# Autodesk Inventor assembly: Factions_Normal
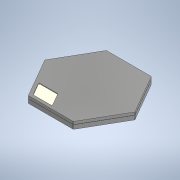
[picture p0: Inventor's stored thumbnail of the model, 180x180]
Saved by Autodesk Inventor 2021 (Build 250183000, 183)
## iProperties
Created: 2023-03-16
Part Number: Factions_Normal
Document SubType Name: Assembly
Designer: Bradley
Author: Bradley
## Documents named in this file (7)
- C:\Users\Bradley\Git\TI4\Factions\Factions_Normal.iam
- C:\Users\Bradley\Git\TI4\Components\Hex_Single.ipt
- C:\Users\Bradley\Git\TI4\Components\FactionCards_All.ipt
- C:\Users\Bradley\Git\TI4\Factions\Factions_Lid.ipt
- C:\Users\Bradley\Git\TI4\Factions\Factions_Base.ipt
- C:\Users\Bradley\Git\TI4\Components\CommandToken_Single.ipt
- C:\Users\Bradley\Git\TI4\Components\ControlMarker_Single.ipt
## Components (37 placed, 6 different names)
1. Factions_Base:1 — Mate:1, Flush:1, Flush:2, Mate:2, Mate:3, Mate:4, Mate:5, Mate:8, Mate:11, Mate:12, Mate:13, Mate:30, Mate:31, Mate:32, Mate:33, Mate:35, Mate:36, Mate:37, Mate:39, Mate:41, Mate:42, Mate:43, Mate:44, Mate:45, Mate:47, Mate:48, Mate:49, Mate:50, Mate:52, Mate:53, Mate:56, Mate:59, Mate:61
2. Factions_Lid:1 — Mate:1, Flush:1, Flush:2
3. CommandToken_Single:1 — Mate:6, Flush:6, Flush:8, Mate:8, Mate:12, Mate:13, Mate:60
4. CommandToken_Single:10 — Mate:36, Mate:37, Mate:38, Mate:40
5. CommandToken_Single:11
6. CommandToken_Single:12
7. CommandToken_Single:13 — Mate:39, Mate:40, Mate:41
8. CommandToken_Single:14
9. CommandToken_Single:15
10. CommandToken_Single:16 — Mate:58, Mate:61, Flush:47
11. CommandToken_Single:2 — Mate:6, Mate:7, Flush:5, Flush:6, Flush:7, Flush:8
12. CommandToken_Single:3 — Mate:7, Flush:5, Flush:7
13. CommandToken_Single:4 — Mate:30, Mate:31, Mate:32, Mate:34
14. CommandToken_Single:5
15. CommandToken_Single:6
16. CommandToken_Single:7 — Mate:33, Mate:34, Mate:35, Mate:38
17. CommandToken_Single:8
18. CommandToken_Single:9
19. ControlMarker_Single:1 — Mate:9, Flush:9, Flush:11, Mate:11, Mate:42, Mate:43, Mate:46
20. ControlMarker_Single:10 — Mate:47, Mate:48, Mate:49, Mate:51
21. ControlMarker_Single:11
22. ControlMarker_Single:12
23. ControlMarker_Single:13 — Mate:50, Mate:51, Mate:52, Mate:54
24. ControlMarker_Single:14
25. ControlMarker_Single:15
26. ControlMarker_Single:16 — Mate:56, Mate:57, Flush:45, Flush:46, Mate:59, Mate:60
27. ControlMarker_Single:17 — Mate:57, Mate:58, Flush:45, Flush:46, Flush:47
28. ControlMarker_Single:2 — Mate:9, Mate:10, Flush:9, Flush:10, Flush:11, Flush:12
29. ControlMarker_Single:3 — Mate:10, Flush:10, Flush:12
30. ControlMarker_Single:4 — Mate:53, Mate:54, Mate:55
31. ControlMarker_Single:5
32. ControlMarker_Single:6
33. ControlMarker_Single:7 — Mate:44, Mate:45, Mate:46, Mate:55
34. ControlMarker_Single:8
35. ControlMarker_Single:9
36. FactionCards_All:1 — Mate:3, Mate:4, Mate:5
37. Hex_Single:1 — Mate:2, Flush:3, Flush:4
## Relationships (108: Mate 61, Flush 47)
- Mate:1: Factions_Base:1 ↔ Factions_Lid:1
- Flush:1: Factions_Base:1 ↔ Factions_Lid:1
- Flush:2: Factions_Base:1 ↔ Factions_Lid:1
- Mate:2: Factions_Base:1 ↔ Hex_Single:1
- Flush:3: Hex_Single:1
- Flush:4: Hex_Single:1
- Mate:3: Factions_Base:1 ↔ FactionCards_All:1
- Mate:4 (0.5 mm): Factions_Base:1 ↔ FactionCards_All:1
- Mate:5 (0.5 mm): Factions_Base:1 ↔ FactionCards_All:1
- Mate:6: CommandToken_Single:1 ↔ CommandToken_Single:2
- Mate:7: CommandToken_Single:2 ↔ CommandToken_Single:3
- Flush:5: CommandToken_Single:2 ↔ CommandToken_Single:3
- Flush:6: CommandToken_Single:1 ↔ CommandToken_Single:2
- Flush:7: CommandToken_Single:2 ↔ CommandToken_Single:3
- Flush:8: CommandToken_Single:1 ↔ CommandToken_Single:2
- Mate:8: Factions_Base:1 ↔ CommandToken_Single:1
- Mate:9: ControlMarker_Single:1 ↔ ControlMarker_Single:2
- Mate:10: ControlMarker_Single:2 ↔ ControlMarker_Single:3
- Flush:9: ControlMarker_Single:1 ↔ ControlMarker_Single:2
- Flush:10: ControlMarker_Single:2 ↔ ControlMarker_Single:3
- Flush:11: ControlMarker_Single:1 ↔ ControlMarker_Single:2
- Flush:12: ControlMarker_Single:2 ↔ ControlMarker_Single:3
- Mate:11: Factions_Base:1 ↔ ControlMarker_Single:1
- Mate:12 (0.5 mm): Factions_Base:1 ↔ CommandToken_Single:1
- Mate:13 (0.5 mm): Factions_Base:1 ↔ CommandToken_Single:1
- [Mate]: CommandToken_Single:4 ↔ CommandToken_Single:5
- [Mate]: CommandToken_Single:5 ↔ CommandToken_Single:6
- [Flush]: CommandToken_Single:5 ↔ CommandToken_Single:6
- [Flush]: CommandToken_Single:4 ↔ CommandToken_Single:5
- [Flush]: CommandToken_Single:5 ↔ CommandToken_Single:6
- [Flush]: CommandToken_Single:4 ↔ CommandToken_Single:5
- [Mate]: CommandToken_Single:7 ↔ CommandToken_Single:8
- [Mate]: CommandToken_Single:8 ↔ CommandToken_Single:9
- [Flush]: CommandToken_Single:8 ↔ CommandToken_Single:9
- [Flush]: CommandToken_Single:7 ↔ CommandToken_Single:8
- [Flush]: CommandToken_Single:8 ↔ CommandToken_Single:9
- [Flush]: CommandToken_Single:7 ↔ CommandToken_Single:8
- [Mate]: CommandToken_Single:10 ↔ CommandToken_Single:11
- [Mate]: CommandToken_Single:11 ↔ CommandToken_Single:12
- [Flush]: CommandToken_Single:11 ↔ CommandToken_Single:12
- [Flush]: CommandToken_Single:10 ↔ CommandToken_Single:11
- [Flush]: CommandToken_Single:11 ↔ CommandToken_Single:12
- [Flush]: CommandToken_Single:10 ↔ CommandToken_Single:11
- [Mate]: CommandToken_Single:13 ↔ CommandToken_Single:14
- [Mate]: CommandToken_Single:14 ↔ CommandToken_Single:15
- [Flush]: CommandToken_Single:14 ↔ CommandToken_Single:15
- [Flush]: CommandToken_Single:13 ↔ CommandToken_Single:14
- [Flush]: CommandToken_Single:14 ↔ CommandToken_Single:15
- [Flush]: CommandToken_Single:13 ↔ CommandToken_Single:14
- [Mate]: ControlMarker_Single:4 ↔ ControlMarker_Single:5
- [Mate]: ControlMarker_Single:5 ↔ ControlMarker_Single:6
- [Flush]: ControlMarker_Single:4 ↔ ControlMarker_Single:5
- [Flush]: ControlMarker_Single:5 ↔ ControlMarker_Single:6
- [Flush]: ControlMarker_Single:4 ↔ ControlMarker_Single:5
- [Flush]: ControlMarker_Single:5 ↔ ControlMarker_Single:6
- [Mate]: ControlMarker_Single:7 ↔ ControlMarker_Single:8
- [Mate]: ControlMarker_Single:8 ↔ ControlMarker_Single:9
- [Flush]: ControlMarker_Single:7 ↔ ControlMarker_Single:8
- [Flush]: ControlMarker_Single:8 ↔ ControlMarker_Single:9
- [Flush]: ControlMarker_Single:7 ↔ ControlMarker_Single:8
- [Flush]: ControlMarker_Single:8 ↔ ControlMarker_Single:9
- [Mate]: ControlMarker_Single:10 ↔ ControlMarker_Single:11
- [Mate]: ControlMarker_Single:11 ↔ ControlMarker_Single:12
- [Flush]: ControlMarker_Single:10 ↔ ControlMarker_Single:11
- [Flush]: ControlMarker_Single:11 ↔ ControlMarker_Single:12
- [Flush]: ControlMarker_Single:10 ↔ ControlMarker_Single:11
- [Flush]: ControlMarker_Single:11 ↔ ControlMarker_Single:12
- [Mate]: ControlMarker_Single:13 ↔ ControlMarker_Single:14
- [Mate]: ControlMarker_Single:14 ↔ ControlMarker_Single:15
- [Flush]: ControlMarker_Single:13 ↔ ControlMarker_Single:14
- [Flush]: ControlMarker_Single:14 ↔ ControlMarker_Single:15
- [Flush]: ControlMarker_Single:13 ↔ ControlMarker_Single:14
- [Flush]: ControlMarker_Single:14 ↔ ControlMarker_Single:15
- Mate:30: Factions_Base:1 ↔ CommandToken_Single:4
- Mate:31 (0.5 mm): Factions_Base:1 ↔ CommandToken_Single:4
- Mate:32 (0.5 mm): Factions_Base:1 ↔ CommandToken_Single:4
- Mate:33: Factions_Base:1 ↔ CommandToken_Single:7
- Mate:34 (0.5 mm): CommandToken_Single:4 ↔ CommandToken_Single:7
- Mate:35 (0.5 mm): Factions_Base:1 ↔ CommandToken_Single:7
- Mate:36: Factions_Base:1 ↔ CommandToken_Single:10
- Mate:37 (0.5 mm): Factions_Base:1 ↔ CommandToken_Single:10
- Mate:38 (0.5 mm): CommandToken_Single:10 ↔ CommandToken_Single:7
- Mate:39: Factions_Base:1 ↔ CommandToken_Single:13
- Mate:40 (0.5 mm): CommandToken_Single:10 ↔ CommandToken_Single:13
- Mate:41 (0.5 mm): Factions_Base:1 ↔ CommandToken_Single:13
- Mate:42 (0.5 mm): Factions_Base:1 ↔ ControlMarker_Single:1
- Mate:43 (0.5 mm): Factions_Base:1 ↔ ControlMarker_Single:1
- Mate:44: Factions_Base:1 ↔ ControlMarker_Single:7
- Mate:45 (0.5 mm): Factions_Base:1 ↔ ControlMarker_Single:7
- Mate:46 (0.5 mm): ControlMarker_Single:1 ↔ ControlMarker_Single:7
- Mate:47: Factions_Base:1 ↔ ControlMarker_Single:10
- Mate:48 (0.5 mm): Factions_Base:1 ↔ ControlMarker_Single:10
- Mate:49 (0.5 mm): Factions_Base:1 ↔ ControlMarker_Single:10
- Mate:50: Factions_Base:1 ↔ ControlMarker_Single:13
- Mate:51 (0.5 mm): ControlMarker_Single:10 ↔ ControlMarker_Single:13
- Mate:52 (0.5 mm): Factions_Base:1 ↔ ControlMarker_Single:13
- Mate:53: Factions_Base:1 ↔ ControlMarker_Single:4
- Mate:54 (0.5 mm): ControlMarker_Single:13 ↔ ControlMarker_Single:4
- Mate:55: ControlMarker_Single:4 ↔ ControlMarker_Single:7
- Mate:56: Factions_Base:1 ↔ ControlMarker_Single:16
- Mate:57: ControlMarker_Single:16 ↔ ControlMarker_Single:17
- Mate:58: CommandToken_Single:16 ↔ ControlMarker_Single:17
- Flush:45: ControlMarker_Single:16 ↔ ControlMarker_Single:17
- Flush:46: ControlMarker_Single:16 ↔ ControlMarker_Single:17
- Mate:59 (0.5 mm): Factions_Base:1 ↔ ControlMarker_Single:16
- Mate:60 (0.5 mm): CommandToken_Single:1 ↔ ControlMarker_Single:16
- Mate:61 (0.5 mm): Factions_Base:1 ↔ CommandToken_Single:16
- Flush:47: CommandToken_Single:16 ↔ ControlMarker_Single:17
## Named parameters: d25_d14 = 0 mm, d26_d9 = 0 mm, d27_d10 = 0 mm, d28_d11 = 0 mm, d29_d12 = 0 mm, d30_d13 = 0 mm, d31_d14 = 0 mm, d32_d9 = 0 mm, d33_d10 = 0 mm, d34_d11 = 0 mm, d35_d12 = 0 mm, d36_d13 = 0 mm, d37_d14 = 0 mm, d38_d9 = 0 mm, d39_d10 = 0 mm, d40_d11 = 0 mm, d41_d12 = 0 mm, d42_d13 = 0 mm, d43_d14 = 0 mm, d44_d9 = 0 mm, d45_d10 = 0 mm, d46_d11 = 0 mm, d47_d12 = 0 mm, d48_d13 = 0 mm, d49_d16 = 0 mm, d50_d17 = 0 mm, d51_d18 = 0 mm, d52_d19 = 0 mm, d53_d20 = 0 mm, d54_d21 = 0 mm, d55_d16 = 0 mm, d56_d17 = 0 mm, d57_d18 = 0 mm, d58_d19 = 0 mm, d59_d20 = 0 mm, d60_d21 = 0 mm, d61_d16 = 0 mm, d62_d17 = 0 mm, d63_d18 = 0 mm, d64_d19 = 0 mm, d65_d20 = 0 mm, d66_d21 = 0 mm, d67_d16 = 0 mm, d68_d17 = 0 mm, d69_d18 = 0 mm, d70_d19 = 0 mm, d71_d20 = 0 mm, d72_d21 = 0 mm
